# Autodesk Inventor assembly: Assemblyclaw pulley idea
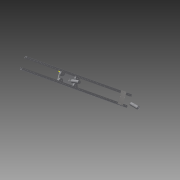
[picture p0: Inventor's stored thumbnail of the model, 180x180]
Saved by Autodesk Inventor 2015 (Build 190159000, 159)
## iProperties
Created: 2015-01-28
Part Number: Assemblyclaw pulley idea
Document SubType Name: Assembly
Designer: chapale16
Author: chapale16
Title: \\lhssvr02\Homedirs\Robotics Club\CAD Model 2015\claw\Assemblyclaw pulley idea.stp
Creation Date: 2015-01-27
Sending System: Autodesk Inventor 2015
Preprocessor: ST-DEVELOPER v15.6
## Documents named in this file (10)
- \\lhssvr02\Homedirs\Robotics Club\CAD Model 2015\claw\Assemblyclaw pulley idea.iam
- \\lhssvr02\Homedirs\Robotics Club\CAD Model 2015\claw\trolley plate.ipt
- \\lhssvr02\Homedirs\Robotics Club\CAD Model 2015\claw\wheel.ipt
- \\lhssvr02\Homedirs\Robotics Club\CAD Model 2015\claw\.313 peg.ipt
- \\lhssvr02\Homedirs\Robotics Club\CAD Model 2015\claw\c hannel.ipt
- \\lhssvr02\Homedirs\Robotics Club\CAD Model 2015\claw\motor.ipt
- \\lhssvr02\Homedirs\Robotics Club\CAD Model 2015\claw\#6 screw.ipt
- \\lhssvr02\Homedirs\Robotics Club\CAD Model 2015\claw\motor plate.ipt
- \\lhssvr02\Homedirs\Robotics Club\CAD Model 2015\claw\.25 peg.ipt
- \\lhssvr02\Homedirs\Robotics Club\CAD Model 2015\claw\Imported Components\PG-71-am-0914\PG-71-am-0914.ipt
## Components (24 placed, 9 different names)
1. trolley plate:1
2. wheel:1
3. wheel:2
4. wheel:3
5. wheel:4
6. .313 peg:1
7. .313 peg:2
8. .313 peg:3
9. .313 peg:4
10. c hannel:1
11. c hannel:2 — Tangent:1, Flush:1
12. motor:1
13. #6 screw:1
14. #6 screw:2
15. #6 screw:3
16. #6 screw:4
17. motor plate:1 — Insert:1, Insert:2, Insert:3, Insert:4, Insert:5, Insert:6
18. .25 peg:1 — Insert:2
19. .25 peg:2 — Insert:3, Tangent:1, Flush:1
20. .25 peg:3 — Insert:4
21. .25 peg:4 — Insert:1
22. .25 peg:5 — Insert:6
23. .25 peg:6 — Insert:5
24. PG-71-am-0914:1
## Relationships (8: Insert 6, Tangent 1, Flush 1)
- Insert:1: motor plate:1 ↔ .25 peg:4
- Insert:2: motor plate:1 ↔ .25 peg:1
- Insert:3: motor plate:1 ↔ .25 peg:2
- Insert:4: motor plate:1 ↔ .25 peg:3
- Insert:5: motor plate:1 ↔ .25 peg:6
- Insert:6: motor plate:1 ↔ .25 peg:5
- Tangent:1: c hannel:2 ↔ .25 peg:2
- Flush:1: c hannel:2 ↔ .25 peg:2
